# Autodesk Inventor assembly: testAssembly
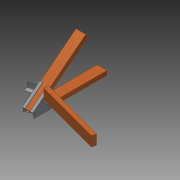
[picture p0: Inventor's stored thumbnail of the model, 180x180]
Saved by Autodesk Inventor 2014 (Build 180170000, 170)
## iProperties
Created: 2015-03-20
Part Number: testAssembly
Document SubType Name: Assembly
Designer: ddeboer
Author: ddeboer
## Documents named in this file (4)
- C:\Users\ddeboer\Desktop\hera-cad\endcaps\testAssembly.iam
- C:\Users\ddeboer\Desktop\hera-cad\endcaps\2by4.ipt
- C:\Users\ddeboer\Desktop\hera-cad\endcaps\fabrication model end cap left-1.iam
- C:\Users\ddeboer\Desktop\hera-cad\endcaps\fabrication model end cap right-1.iam
## Components (5 placed, 3 different names)
1. 2by4:1 — Mate:1, Mate:4, Mate:5
2. fabrication model end cap left-1:1 [sub-assembly] — Mate:5, Mate:6, Flush:1
3. fabrication model end cap right-1:1 [sub-assembly] — Mate:1, Mate:2, Mate:3, Mate:4, Mate:7, Mate:8, Flush:1
4. 2by4:2 — Mate:2, Mate:3, Mate:6
5. 2by4:3 — Mate:7, Mate:8
## Relationships (9: Mate 8, Flush 1)
- Mate:1: 2by4:1 ↔ fabrication model end cap right-1:1
- Mate:2: fabrication model end cap right-1:1 ↔ 2by4:2
- Mate:3: fabrication model end cap right-1:1 ↔ 2by4:2
- Mate:4: 2by4:1 ↔ fabrication model end cap right-1:1
- Mate:5: 2by4:1 ↔ fabrication model end cap left-1:1
- Mate:6: fabrication model end cap left-1:1 ↔ 2by4:2
- Mate:7: fabrication model end cap right-1:1 ↔ 2by4:3
- Mate:8: fabrication model end cap right-1:1 ↔ 2by4:3
- Flush:1: fabrication model end cap left-1:1 ↔ fabrication model end cap right-1:1
